# Autodesk Inventor assembly: E002-Piston
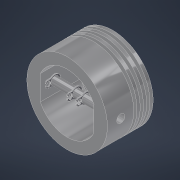
[picture p0: Inventor's stored thumbnail of the model, 180x180]
Saved by Autodesk Inventor 2021.3 (Build 253353000, 353)
## iProperties
Company: HES-SO
Created: 2022-03-31
Part Number: E002-Piston
Document SubType Name: Assembly
Designer: HER & ZAE
Mass: 16.0937 g
Surface Area: 54.7339 cm^2
Volume: 5.9686 cm^3
Density: 2.6964 g/cm^3
Author: HER & ZAE
## Documents named in this file (4)
- C:\Users\remi\OneDrive\Documents\Cours\05-HEVS\S2fb\mechanic\CCo\project\Compressor\E002-Piston.iam
- C:\Users\remi\OneDrive\Documents\Cours\05-HEVS\S2fb\mechanic\CCo\project\Compressor\P003-Corps_piston.ipt
- C:\Users\remi\OneDrive\Documents\Cours\05-HEVS\S2fb\mechanic\CCo\project\Compressor\P005-Axe_piston.ipt
- C:\Users\remi\OneDrive\Documents\Cours\05-HEVS\S2fb\mechanic\CCo\project\Compressor\Circlips\ungespannt_61799403.ipt
## Components (6 placed, 3 different names)
1. P003-Corps_piston:1 — Mate:1, Flush:1
2. P005-Axe_piston:1 — Mate:1, Flush:1, Mate:2, Mate:3, Mate:4, Mate:5, Mate:6, Mate:7, Mate:8, Mate:9
3. ungespannt_61799403:1 — Mate:2, Mate:4
4. ungespannt_61799403:2 — Mate:3, Mate:5
5. ungespannt_61799403:4 — Mate:6, Mate:9
6. ungespannt_61799403:5 — Mate:7, Mate:8
## Relationships (10: Mate 9, Flush 1)
- Mate:1: P003-Corps_piston:1 ↔ P005-Axe_piston:1
- Flush:1: P003-Corps_piston:1 ↔ P005-Axe_piston:1
- Mate:2: P005-Axe_piston:1 ↔ ungespannt_61799403:1
- Mate:3: P005-Axe_piston:1 ↔ ungespannt_61799403:2
- Mate:4: P005-Axe_piston:1 ↔ ungespannt_61799403:1
- Mate:5: P005-Axe_piston:1 ↔ ungespannt_61799403:2
- Mate:6: P005-Axe_piston:1 ↔ ungespannt_61799403:4
- Mate:7: P005-Axe_piston:1 ↔ ungespannt_61799403:5
- Mate:8: P005-Axe_piston:1 ↔ ungespannt_61799403:5
- Mate:9: P005-Axe_piston:1 ↔ ungespannt_61799403:4
